# Autodesk Inventor assembly: 1x3 button assembly
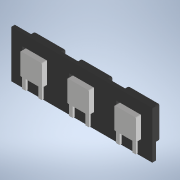
[picture p0: Inventor's stored thumbnail of the model, 180x180]
Saved by Autodesk Inventor 2022 (Build 260153000, 153)
## iProperties
Created: 2022-06-11
Part Number: 1x3 button assembly
Document SubType Name: Assembly
Designer: alecw
Author: alecw
## Documents named in this file (3)
- C:\aw_gd\Coding and Projects\smart home\smart-deadbolt\3D Modelling\1x3 button assembly.iam
- C:\aw_gd\Coding and Projects\smart home\smart-deadbolt\3D Modelling\single 6x6x5 button.ipt
- C:\aw_gd\Coding and Projects\smart home\smart-deadbolt\3D Modelling\1x3 button cover.ipt
## Components (4 placed, 2 different names)
1. 1x3 button cover:1 — Mate:1, Mate:2, Mate:3
2. single 6x6x5 button:1 — Mate:1, Mate:2, Mate:3
3. single 6x6x5 button:2
4. single 6x6x5 button:3
## Component patterns: (3 elements, first: single 6x6x5 button:1)
## Relationships (3: Mate 3)
- Mate:1: 1x3 button cover:1 ↔ single 6x6x5 button:1
- Mate:2 (0.4 mm): 1x3 button cover:1 ↔ single 6x6x5 button:1
- Mate:3 (0.4 mm): 1x3 button cover:1 ↔ single 6x6x5 button:1
